# Autodesk Inventor assembly: Full Assembly
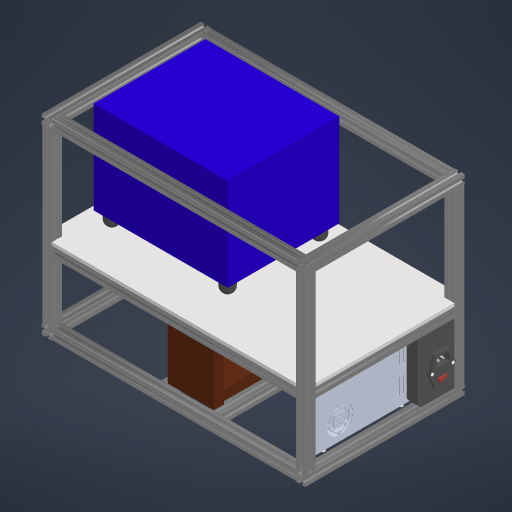
[picture p0: Inventor's stored thumbnail of the model, 512x512]
Saved by Autodesk Inventor 2024.3 (Build 283343000, 343)
## iProperties
Created: 2024-06-11
Part Number: Full Assembly
Document SubType Name: Assembly
Designer: braed
Author: braed
## Documents named in this file (10)
- C:\Users\braed\Documents\Inventor\SPRI\Full Assembly.iam
- C:\Users\braed\Documents\Inventor\SPRI\12in T-Slot.ipt
- C:\Users\braed\Documents\Inventor\SPRI\18.4in T-Slot.ipt
- C:\Users\braed\Documents\Inventor\SPRI\12.95in T-Slot.ipt
- C:\Users\braed\Documents\Inventor\SPRI\10.425in T-Slot.ipt
- C:\Users\braed\Documents\Inventor\SPRI\Magnet.ipt
- C:\Users\braed\Documents\Inventor\SPRI\Pump.ipt
- C:\Users\braed\Documents\Inventor\SPRI\PXie-1083.ipt
- C:\Users\braed\Documents\Inventor\SPRI\Sheet.ipt
- C:\Users\braed\Documents\Inventor\SPRI\Ender 3 PSU.iam
## Components (24 placed, 9 different names)
1. 12in T-Slot:1 — Mate:2, Flush:5, Flush:6, Flush:7, Flush:8, Flush:16, Mate:11
2. 12in T-Slot:4 — Mate:1, Flush:3, Flush:4, Mate:3, Mate:46
3. 18.4in T-Slot:3 — Mate:3, Flush:7, Flush:8, Flush:15
4. 18.4in T-Slot:4 — Mate:1, Flush:3, Flush:4, Mate:2, Flush:5, Flush:6, Mate:45
5. 12in T-Slot:5 — Flush:16, Mate:9, Flush:21, Flush:22, Mate:10, Flush:23, Flush:24
6. 12in T-Slot:6 — Mate:7, Flush:17, Flush:18, Mate:8, Flush:19, Flush:20, Mate:27
7. 18.4in T-Slot:5 — Flush:15, Mate:16, Mate:32
8. 18.4in T-Slot:6 — Mate:23, Flush:44, Mate:24, Flush:45
9. 12.95in T-Slot:1 — Mate:8, Flush:19, Flush:20
10. 12.95in T-Slot:2 — Mate:9, Flush:21, Flush:22, Mate:13, Flush:26, Mate:14, Flush:27, Mate:43
11. 12.95in T-Slot:3 — Mate:10, Flush:23, Flush:24, Mate:11, Mate:41
12. 12.95in T-Slot:4 — Mate:7, Flush:17, Flush:18, Mate:12, Flush:25, Mate:15, Flush:28
13. 10.425in T-Slot:1 — Mate:12, Flush:25, Flush:29, Flush:30, Mate:30
14. 10.425in T-Slot:2 — Mate:13, Flush:26, Flush:31, Mate:31, Flush:60, Mate:44, Flush:61
15. 18.4in T-Slot:7 — Mate:14, Flush:27, Flush:30, Mate:28, Mate:29, Flush:47, Flush:48
16. 18.4in T-Slot:8 — Mate:15, Flush:28, Flush:29, Flush:31, Mate:16, Mate:40
17. 10.425in T-Slot:3 — Mate:24, Flush:45, Mate:25
18. 10.425in T-Slot:4 — Mate:23, Flush:44, Mate:25, Mate:27, Flush:62, Mate:47
19. Magnet:1 — Mate:32, Flush:62, Mate:47
20. Pump:1 — Mate:28, Flush:48, Mate:30
21. Pump:2 — Mate:29, Flush:47, Mate:31
22. PXie-1083:1 — Mate:42, Mate:45, Mate:46
23. Sheet:1 — Mate:40, Flush:60, Mate:41, Mate:42
24. Ender 3 PSU:1 [sub-assembly] — Mate:43, Mate:44, Flush:61
## Relationships (69: Flush 36, Mate 33)
- Mate:1: 12in T-Slot:4 ↔ 18.4in T-Slot:4
- Flush:3: 12in T-Slot:4 ↔ 18.4in T-Slot:4
- Flush:4: 12in T-Slot:4 ↔ 18.4in T-Slot:4
- Mate:2: 12in T-Slot:1 ↔ 18.4in T-Slot:4
- Flush:5: 12in T-Slot:1 ↔ 18.4in T-Slot:4
- Flush:6: 12in T-Slot:1 ↔ 18.4in T-Slot:4
- Mate:3: 12in T-Slot:4 ↔ 18.4in T-Slot:3
- Flush:7: 12in T-Slot:1 ↔ 18.4in T-Slot:3
- Flush:8: 12in T-Slot:1 ↔ 18.4in T-Slot:3
- [Mate]: 12in T-Slot:6 ↔ 18.4in T-Slot:6
- [Flush]: 12in T-Slot:6 ↔ 18.4in T-Slot:6
- [Flush]: 12in T-Slot:6 ↔ 18.4in T-Slot:6
- [Mate]: 12in T-Slot:5 ↔ 18.4in T-Slot:6
- [Flush]: 12in T-Slot:5 ↔ 18.4in T-Slot:6
- [Flush]: 12in T-Slot:5 ↔ 18.4in T-Slot:6
- [Mate]: 12in T-Slot:6 ↔ 18.4in T-Slot:5
- [Flush]: 12in T-Slot:5 ↔ 18.4in T-Slot:5
- [Flush]: 12in T-Slot:5 ↔ 18.4in T-Slot:5
- Flush:15: 18.4in T-Slot:3 ↔ 18.4in T-Slot:5
- Flush:16: 12in T-Slot:1 ↔ 12in T-Slot:5
- Mate:7: 12in T-Slot:6 ↔ 12.95in T-Slot:4
- Flush:17: 12in T-Slot:6 ↔ 12.95in T-Slot:4
- Flush:18: 12in T-Slot:6 ↔ 12.95in T-Slot:4
- Mate:8: 12in T-Slot:6 ↔ 12.95in T-Slot:1
- Flush:19: 12in T-Slot:6 ↔ 12.95in T-Slot:1
- Flush:20: 12in T-Slot:6 ↔ 12.95in T-Slot:1
- Mate:9: 12in T-Slot:5 ↔ 12.95in T-Slot:2
- Flush:21: 12in T-Slot:5 ↔ 12.95in T-Slot:2
- Flush:22: 12in T-Slot:5 ↔ 12.95in T-Slot:2
- Mate:10: 12in T-Slot:5 ↔ 12.95in T-Slot:3
- Flush:23: 12in T-Slot:5 ↔ 12.95in T-Slot:3
- Flush:24: 12in T-Slot:5 ↔ 12.95in T-Slot:3
- Mate:11: 12in T-Slot:1 ↔ 12.95in T-Slot:3
- Mate:12: 12.95in T-Slot:4 ↔ 10.425in T-Slot:1
- Flush:25: 12.95in T-Slot:4 ↔ 10.425in T-Slot:1
- Mate:13: 12.95in T-Slot:2 ↔ 10.425in T-Slot:2
- Flush:26: 12.95in T-Slot:2 ↔ 10.425in T-Slot:2
- Mate:14: 12.95in T-Slot:2 ↔ 18.4in T-Slot:7
- Flush:27: 12.95in T-Slot:2 ↔ 18.4in T-Slot:7
- Mate:15: 12.95in T-Slot:4 ↔ 18.4in T-Slot:8
- Flush:28: 12.95in T-Slot:4 ↔ 18.4in T-Slot:8
- Flush:29: 10.425in T-Slot:1 ↔ 18.4in T-Slot:8
- Flush:30: 10.425in T-Slot:1 ↔ 18.4in T-Slot:7
- Flush:31: 10.425in T-Slot:2 ↔ 18.4in T-Slot:8
- Mate:16 (117.475 mm): 18.4in T-Slot:5 ↔ 18.4in T-Slot:8
- Mate:23: 18.4in T-Slot:6 ↔ 10.425in T-Slot:4
- Flush:44: 18.4in T-Slot:6 ↔ 10.425in T-Slot:4
- Mate:24: 18.4in T-Slot:6 ↔ 10.425in T-Slot:3
- Flush:45: 18.4in T-Slot:6 ↔ 10.425in T-Slot:3
- Mate:25 (74.4 mm): 10.425in T-Slot:3 ↔ 10.425in T-Slot:4
- Mate:27 (189.55 mm): 12in T-Slot:6 ↔ 10.425in T-Slot:4
- Mate:28: 18.4in T-Slot:7 ↔ Pump:1
- Mate:29: 18.4in T-Slot:7 ↔ Pump:2
- Flush:47 (3.556 mm): 18.4in T-Slot:7 ↔ Pump:2
- Flush:48 (-3.556 mm): 18.4in T-Slot:7 ↔ Pump:1
- Mate:30 (25.4 mm): 10.425in T-Slot:1 ↔ Pump:1
- Mate:31 (38.1 mm): 10.425in T-Slot:2 ↔ Pump:2
- Mate:32: 18.4in T-Slot:5 ↔ Magnet:1
- Mate:40: 18.4in T-Slot:8 ↔ Sheet:1
- Flush:60: 10.425in T-Slot:2 ↔ Sheet:1
- Mate:41: 12.95in T-Slot:3 ↔ Sheet:1
- Mate:42: PXie-1083:1 ↔ Sheet:1
- Mate:43: 12.95in T-Slot:2 ↔ Ender 3 PSU:1
- Mate:44: 10.425in T-Slot:2 ↔ Ender 3 PSU:1
- Flush:61: 10.425in T-Slot:2 ↔ Ender 3 PSU:1
- Mate:45 (3.175 mm): 18.4in T-Slot:4 ↔ PXie-1083:1
- Mate:46 (12.7 mm): 12in T-Slot:4 ↔ PXie-1083:1
- Flush:62 (12.5 mm): 10.425in T-Slot:4 ↔ Magnet:1
- Mate:47: 10.425in T-Slot:4 ↔ Magnet:1
## Named parameters: d9_d0 = 0 mm, d10_d1 = 0 mm, d11_d2 = 0 mm, d12_d3 = 0 mm, d13_d4 = 0 mm, d14_d5 = 0 mm, d15_d6 = 0 mm, d16_d7 = 0 mm, d17_d8 = 0 mm
